# Autodesk Inventor assembly: Wagomount_Construction
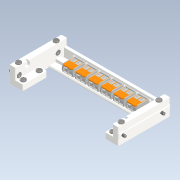
[picture p0: Inventor's stored thumbnail of the model, 180x180]
Saved by Autodesk Inventor 2022.1 (Build 261234020, 234B)
## iProperties
Created: 2022-07-24
Part Number: Wagomount_Construction
Document SubType Name: Assembly
Designer: Rama
Author: Rama
## Documents named in this file (5)
- C:\Users\Rama\Desktop\GitHub\Voron-2-Mods\Mandalaroseworks\BedPan\CAD\SRC\Manual_Helpers\Wagomount_Construction.iam
- C:\Users\Rama\Desktop\GitHub\Voron-2-Mods\Mandalaroseworks\BedPan\CAD\SRC\Wagomount\Wagomount.ipt
- C:\Users\Rama\Desktop\Work Priv\Klicky\6x3 Magnet.ipt
- C:\Users\Rama\Downloads\221-412.ipt
- C:\Users\Rama\Desktop\RAMA_SBNG\ToolheadNEW\ContentCenter\de-DE\DIN 912\DIN 912 - M3 x 0,5 x 8 x 6,75.ipt
## Components (19 placed, 4 different names)
1. Wagomount:1 — Passend:1, Passend:2, Passend:3, Passend:4, Passend:5, Passend:6, Passend:7, Passend:8, Passend:9, Passend:10, Passend:11, Passend:12, Passend:13, Passend:14, Passend:15, Passend:16, Passend:17, Passend:18, Passend:19, Passend:20, Passend:21
2. 6x3 Magnet:1 — Passend:3
3. 6x3 Magnet:2 — Passend:2
4. 6x3 Magnet:3 — Passend:4
5. 6x3 Magnet:4 — Passend:1
6. 6x3 Magnet:5 — Passend:6
7. 6x3 Magnet:6 — Passend:7
8. 6x3 Magnet:7 — Passend:8
9. 6x3 Magnet:8 — Passend:5
10. 221-412:1 — Passend:9, Passend:10, Passend:11, Fluchtend:7
11. 221-412:2 — Fluchtend:7, Fluchtend:8, Fluchtend:13, Passend:12, Passend:13
12. 221-412:3 — Fluchtend:8, Fluchtend:9, Fluchtend:13, Fluchtend:14, Fluchtend:16, Passend:14
13. 221-412:4 — Fluchtend:9, Fluchtend:14, Fluchtend:17, Passend:15
14. 221-412:6 — Fluchtend:12, Fluchtend:16, Passend:17
15. 221-412:7 — Fluchtend:12, Fluchtend:17, Passend:16
16. DIN 912 - ersetzt durch DIN EN ISO 4762 M3 x 8:1 — Passend:18, Fluchtend:19
17. DIN 912 - ersetzt durch DIN EN ISO 4762 M3 x 8:2 — Passend:19, Fluchtend:19
18. DIN 912 - ersetzt durch DIN EN ISO 4762 M3 x 8:3 — Passend:20, Fluchtend:18
19. DIN 912 - ersetzt durch DIN EN ISO 4762 M3 x 8:4 — Passend:21, Fluchtend:18
## Relationships (37: Mate 21, Flush 16)
- [Flush]: 6x3 Magnet:2 ↔ 6x3 Magnet:3
- [Flush]: 6x3 Magnet:1 ↔ 6x3 Magnet:4
- [Flush]: 6x3 Magnet:3 ↔ 6x3 Magnet:4
- Passend:1 [Mate]: Wagomount:1 ↔ 6x3 Magnet:4
- Passend:2 [Mate]: Wagomount:1 ↔ 6x3 Magnet:2
- Passend:3 [Mate]: Wagomount:1 ↔ 6x3 Magnet:1
- Passend:4 [Mate]: Wagomount:1 ↔ 6x3 Magnet:3
- [Flush]: 6x3 Magnet:6 ↔ 6x3 Magnet:7
- [Flush]: 6x3 Magnet:5 ↔ 6x3 Magnet:8
- [Flush]: 6x3 Magnet:7 ↔ 6x3 Magnet:8
- Passend:5 [Mate]: Wagomount:1 ↔ 6x3 Magnet:8
- Passend:6 [Mate]: Wagomount:1 ↔ 6x3 Magnet:5
- Passend:7 [Mate]: Wagomount:1 ↔ 6x3 Magnet:6
- Passend:8 [Mate]: Wagomount:1 ↔ 6x3 Magnet:7
- Passend:9 [Mate]: Wagomount:1 ↔ 221-412:1
- Passend:10 [Mate] (-0.2 mm): Wagomount:1 ↔ 221-412:1
- Passend:11 [Mate]: Wagomount:1 ↔ 221-412:1
- Fluchtend:7 [Flush]: 221-412:1 ↔ 221-412:2
- Fluchtend:8 [Flush]: 221-412:2 ↔ 221-412:3
- Fluchtend:9 [Flush]: 221-412:3 ↔ 221-412:4
- Fluchtend:12 [Flush]: 221-412:6 ↔ 221-412:7
- Fluchtend:13 [Flush]: 221-412:2 ↔ 221-412:3
- Fluchtend:14 [Flush]: 221-412:3 ↔ 221-412:4
- Fluchtend:16 [Flush]: 221-412:3 ↔ 221-412:6
- Fluchtend:17 [Flush]: 221-412:4 ↔ 221-412:7
- Passend:12 [Mate]: Wagomount:1 ↔ 221-412:2
- Passend:13 [Mate] (-0.2 mm): Wagomount:1 ↔ 221-412:2
- Passend:14 [Mate] (-0.2 mm): Wagomount:1 ↔ 221-412:3
- Passend:15 [Mate] (-0.2 mm): Wagomount:1 ↔ 221-412:4
- Passend:16 [Mate] (-0.2 mm): Wagomount:1 ↔ 221-412:7
- Passend:17 [Mate] (-0.2 mm): Wagomount:1 ↔ 221-412:6
- Passend:18 [Mate]: Wagomount:1 ↔ DIN 912 - ersetzt durch DIN EN ISO 4762 M3 x 8:1
- Passend:19 [Mate]: Wagomount:1 ↔ DIN 912 - ersetzt durch DIN EN ISO 4762 M3 x 8:2
- Passend:20 [Mate]: Wagomount:1 ↔ DIN 912 - ersetzt durch DIN EN ISO 4762 M3 x 8:3
- Passend:21 [Mate]: Wagomount:1 ↔ DIN 912 - ersetzt durch DIN EN ISO 4762 M3 x 8:4
- Fluchtend:18 [Flush]: DIN 912 - ersetzt durch DIN EN ISO 4762 M3 x 8:3 ↔ DIN 912 - ersetzt durch DIN EN ISO 4762 M3 x 8:4
- Fluchtend:19 [Flush]: DIN 912 - ersetzt durch DIN EN ISO 4762 M3 x 8:1 ↔ DIN 912 - ersetzt durch DIN EN ISO 4762 M3 x 8:2
## Named parameters: d7_d38 = 0 mm, d8_d39 = 0 mm, d9_d37 = 0 mm
